# Autodesk Inventor assembly: MIRleftMIRright脚一枚1
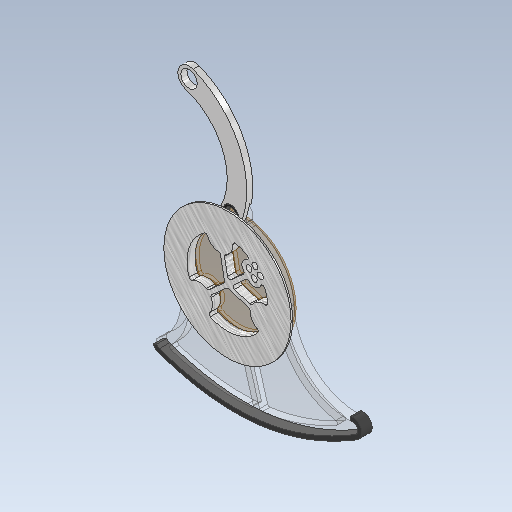
[picture p0: Inventor's stored thumbnail of the model, 512x512]
Saved by Autodesk Inventor 2020.2 (Build 242310000, 310)
## iProperties
Created: 2020-04-13
Part Number: MIRleftMIRright脚一枚1
Document SubType Name: Assembly
Designer: aoyama
Mass: 31.6013 g
Surface Area: 259.988 cm^2
Volume: 17.8864 cm^3
Density: 1.76678 g/cm^3
Author: aoyama
## Documents named in this file (8)
- C:\Users\aoyam\Desktop\SRDC_local\Inventor\二年機\Geminiβ\脚\ネジクランク\MIR達\MIRleftMIRright脚一枚1.iam
- C:\Users\aoyam\Desktop\SRDC_local\Inventor\二年機\Geminiβ\脚\ネジクランク\MIR達\MIRleftMIRrightクランク3t1.ipt
- C:\Users\aoyam\Desktop\SRDC_local\Inventor\二年機\Geminiβ\脚\ネジクランク\MIR達\MIRleftMIRrightクランク4t1.ipt
- C:\Users\aoyam\Desktop\SRDC_local\Inventor\二年機\Geminiβ\汎用部品\MIR達\MIRleftMIRrightベアリングd3D8B4F無.ipt
- C:\Users\aoyam\Desktop\SRDC_local\Inventor\二年機\Geminiβ\脚\ネジクランク\MIR達\MIRleftMIRrightヘッケン改1.ipt
- C:\Users\aoyam\Desktop\SRDC_local\Inventor\二年機\Geminiβ\脚\ネジクランク\MIR達\MIRleftMIRright揺動節1.ipt
- C:\Users\aoyam\Desktop\SRDC_local\Inventor\二年機\Geminiβ\汎用部品\MIR達\MIRleftMIRrightオイレス外径8内径6L2.ipt
- C:\Users\aoyam\Desktop\SRDC_local\Inventor\二年機\Geminiβ\脚\ネジクランク\MIR達\MIRleftMIRright脚ゴム1.ipt
## Components (9 placed, 7 different names)
1. MIRleftMIRrightクランク3t1:1 — 挿入:11, 挿入:15
2. MIRleftMIRrightクランク4t1:1 — 挿入:11, 挿入:8, 挿入:10, 挿入:9, 挿入:14
3. MIRleftMIRrightベアリングd3D8B4F無:1 — 挿入:8
4. MIRleftMIRrightベアリングd3D8B4F無:2 — 挿入:10, 挿入:15
5. MIRleftMIRrightベアリングd3D8B4F無:3 — 挿入:9
6. MIRleftMIRrightヘッケン改1:1 — 挿入:14, 挿入:11, 挿入:13, 挿入:12
7. MIRleftMIRright揺動節1:1 — 挿入:11, 挿入:10
8. MIRleftMIRrightオイレス外径8内径6L2:1 — 挿入:10
9. MIRleftMIRright脚ゴム1:1 — 挿入:13, 挿入:12
## Relationships (10: Insert 10)
- 挿入:11 [Insert]: MIRleftMIRrightクランク3t1:1 ↔ MIRleftMIRrightクランク4t1:1
- 挿入:8 [Insert]: MIRleftMIRrightクランク4t1:1 ↔ MIRleftMIRrightベアリングd3D8B4F無:1
- 挿入:10 [Insert]: MIRleftMIRrightクランク4t1:1 ↔ MIRleftMIRrightベアリングd3D8B4F無:2
- 挿入:15 [Insert]: MIRleftMIRrightクランク3t1:1 ↔ MIRleftMIRrightベアリングd3D8B4F無:2
- 挿入:9 [Insert]: MIRleftMIRrightクランク4t1:1 ↔ MIRleftMIRrightベアリングd3D8B4F無:3
- 挿入:14 [Insert] (0.2 mm): MIRleftMIRrightクランク4t1:1 ↔ MIRleftMIRrightヘッケン改1:1
- 挿入:11 [Insert]: MIRleftMIRrightヘッケン改1:1 ↔ MIRleftMIRright揺動節1:1
- 挿入:13 [Insert]: MIRleftMIRrightヘッケン改1:1 ↔ MIRleftMIRright脚ゴム1:1
- 挿入:12 [Insert]: MIRleftMIRrightヘッケン改1:1 ↔ MIRleftMIRright脚ゴム1:1
- 挿入:10 [Insert]: MIRleftMIRright揺動節1:1 ↔ MIRleftMIRrightオイレス外径8内径6L2:1
